# Autodesk Inventor assembly: bin_assembly
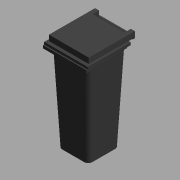
[picture p0: Inventor's stored thumbnail of the model, 180x180]
Saved by Autodesk Inventor 2019 (Build 230136000, 136)
## iProperties
Part Number: bin_assembly
Document SubType Name: Assembly
Designer: Javi
Author: Javi
## Documents named in this file (3)
- D:\MisterBin\base\bin_assembly.iam
- D:\MisterBin\base\bin.ipt
- D:\MisterBin\base\bin_lid.ipt
## Components (2 placed, 2 different names)
1. bin:1 — Rotational:1
2. bin_lid:1 — Rotational:1
## Relationships (1: RevoluteJoint 1)
- Rotational:1 [RevoluteJoint] (10 mm): bin:1 ↔ bin_lid:1
